# Autodesk Inventor assembly: 2_6 assembly
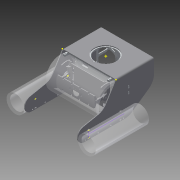
[picture p0: Inventor's stored thumbnail of the model, 180x180]
Saved by Autodesk Inventor 2015 (Build 190159000, 159)
## iProperties
Created: 2015-08-16
Part Number: 2_6 assembly
Document SubType Name: Assembly
Designer: Thomas
Author: Thomas
## Documents named in this file (6)
- C:\Users\Thomas\Google Drive\MSc ROBOTICS\PROJECT\OpenROV\openrov-hardware\CAD_Files_OpenROV_v2_5\2_6 assembly.iam
- C:\Users\Thomas\Google Drive\MSc ROBOTICS\PROJECT\OpenROV\openrov-hardware\CAD_Files_OpenROV_v2_5\battery_Tube.ipt
- C:\Users\Thomas\Google Drive\MSc ROBOTICS\PROJECT\OpenROV\openrov-hardware\CAD_Files_OpenROV_v2_5\E-Chassis_Assemly.iam
- C:\Users\Thomas\Google Drive\MSc ROBOTICS\PROJECT\OpenROV\openrov-hardware\CAD_Files_OpenROV_v2_5\main body assembly.iam
- C:\Users\Thomas\Google Drive\MSc ROBOTICS\PROJECT\OpenROV\openrov-hardware\CAD_Files_OpenROV_v2_5\New_Tube.ipt
- C:\Users\Thomas\Google Drive\MSc ROBOTICS\PROJECT\OpenROV\openrov-hardware\CAD_Files_OpenROV_v2_5\Shell.ipt
## Components (6 placed, 5 different names)
1. Shell:1 — Mate:3, Mate:4, Mate:5, Tangent:3, Mate:7, Tangent:4, Tangent:5, Mate:8, Tangent:6
2. main body assembly:1 [sub-assembly] — Mate:3, Mate:4, Mate:5, Tangent:1, Tangent:2
3. New_Tube:1 — Tangent:1, Tangent:2, Mate:6, Flush:1
4. E-Chassis_Assemly:1 [sub-assembly] — Mate:6, Flush:1
5. battery_Tube:1 — Tangent:5, Mate:8, Tangent:6
6. battery_Tube:2 — Tangent:3, Mate:7, Tangent:4
## Relationships (13: Mate 6, Tangent 6, Flush 1)
- Mate:3: Shell:1 ↔ main body assembly:1
- Mate:4: Shell:1 ↔ main body assembly:1
- Mate:5: Shell:1 ↔ main body assembly:1
- Tangent:1: main body assembly:1 ↔ New_Tube:1
- Tangent:2: main body assembly:1 ↔ New_Tube:1
- Mate:6: New_Tube:1 ↔ E-Chassis_Assemly:1
- Flush:1 (-20 mm): New_Tube:1 ↔ E-Chassis_Assemly:1
- Tangent:3: Shell:1 ↔ battery_Tube:2
- Mate:7: Shell:1 ↔ battery_Tube:2
- Tangent:4: Shell:1 ↔ battery_Tube:2
- Tangent:5: Shell:1 ↔ battery_Tube:1
- Mate:8: Shell:1 ↔ battery_Tube:1
- Tangent:6: Shell:1 ↔ battery_Tube:1
